# Autodesk Inventor assembly: 200-40-BOGIE-CONNECTOR-ASM-01
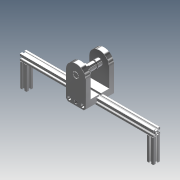
[picture p0: Inventor's stored thumbnail of the model, 180x180]
Saved by Autodesk Inventor 2018.2 (Build 222227000, 227)
## iProperties
Manager: feesmrt
Company: FRANC0R
Created: 2017-12-10
Part Number: 200-40-BOGIE-CONNECTOR-ASM-01
Material: Generisch
Document SubType Name: Assembly
Designer: feesmrt
Project: Rescue Robot
Cost Center: -
Description: Bogie Connector Assembly
Engineer: feesmrt
Authority: feesmrt
Stock Number: 200-40-BOGIE-CONNECTOR-ASM-01
Author: feesmrt
Title: Bogie Connector Assembly
Subject: Rescue Robot
Revision Number: 1
## Documents named in this file (10)
- D:\Programmierung\FRANC0R\CAD\02-Rocker-Bogie-Robot\200-ROCKER-BOGIE\200-40-BOGIE-CONNECTOR-ASM-01.iam
- D:\Programmierung\FRANC0R\CAD\02-Rocker-Bogie-Robot\900-COMPONENTS\900-50-PROFILES\90-50-PROFILES-20x20x400.ipt
- D:\Programmierung\FRANC0R\CAD\02-Rocker-Bogie-Robot\900-COMPONENTS\900-50-PROFILES\90-50-PROFILES-20x20x70.ipt
- D:\Programmierung\FRANC0R\CAD\02-Rocker-Bogie-Robot\200-ROCKER-BOGIE\200-40-BOGIE-CONNECTOR-05.ipt
- D:\Programmierung\FRANC0R\CAD\02-Rocker-Bogie-Robot\200-ROCKER-BOGIE\200-40-BOGIE-CONNECTOR-03.ipt
- D:\Programmierung\FRANC0R\CAD\02-Rocker-Bogie-Robot\200-ROCKER-BOGIE\200-40-BOGIE-CONNECTOR-04.ipt
- D:\Programmierung\FRANC0R\CAD\02-Rocker-Bogie-Robot\900-COMPONENTS\900-40-SCREWS\900-40-SCREWS-DIN7984_M5x25.ipt
- D:\Programmierung\FRANC0R\CAD\02-Rocker-Bogie-Robot\900-COMPONENTS\900-40-SCREWS\900-40-SCREWS-DIN7984_M5x12.ipt
- D:\Programmierung\FRANC0R\CAD\02-Rocker-Bogie-Robot\900-COMPONENTS\900-50-PROFILES\900-50-PROFILES-CONN-N6xM5.ipt
- D:\Programmierung\FRANC0R\CAD\02-Rocker-Bogie-Robot\900-COMPONENTS\900-60-CIRCLIPS\900-60-CIRCLIPS-DIN471-20x1,2.ipt
## Components (19 placed, 9 different names)
1. 200-40-BOGIE-CONNECTOR-05:1 — Passend:6, Passend:7, Fluchtend:7, Passend:8, Passend:9, Passend:10, Passend:45, Passend:46
2. 200-40-BOGIE-CONNECTOR-03:2 — Passend:8, Passend:9, Passend:10, Passend:16, Fluchtend:10, Passend:23, Passend:25, Passend:34, Passend:35
3. 200-40-BOGIE-CONNECTOR-03:1 — Passend:6, Passend:7, Fluchtend:7, Passend:17, Passend:24, Fluchtend:11, Passend:33, Passend:36
4. 90-50-PROFILES-20x20x400:1 — Passend:4, Fluchtend:3, Fluchtend:4, Passend:5, Fluchtend:5, Fluchtend:6, Fluchtend:9, Passend:21, Passend:22
5. 90-50-PROFILES-20x20x70:1 — Passend:5, Fluchtend:5, Fluchtend:6
6. 90-50-PROFILES-20x20x70:2 — Passend:4, Fluchtend:3, Fluchtend:4
7. 200-40-BOGIE-CONNECTOR-04:1 — Passend:17, Passend:21, Passend:24, Fluchtend:11, Passend:29, Passend:30, Passend:31, Passend:32, Passend:39, Passend:40, Winkel:1, Winkel:2
8. 200-40-BOGIE-CONNECTOR-04:2 — Passend:16, Passend:22, Fluchtend:10, Passend:23, Passend:26, Passend:27, Passend:28, Passend:37, Passend:38, Winkel:3, Winkel:4
9. 900-40-SCREWS-DIN7984_M5x25:1 — Passend:25, Passend:26, Passend:41
10. 900-40-SCREWS-DIN7984_M5x25:2 — Passend:27, Passend:28, Passend:42
11. 900-40-SCREWS-DIN7984_M5x25:3 — Passend:30, Passend:32, Passend:44
12. 900-40-SCREWS-DIN7984_M5x25:4 — Passend:29, Passend:31, Passend:43
13. 900-40-SCREWS-DIN7984_M5x12:1 — Passend:33, Passend:36
14. 900-40-SCREWS-DIN7984_M5x12:2 — Passend:34, Passend:35
15. 900-50-PROFILES-CONN-N6xM5:1 — Passend:37, Passend:42, Winkel:4
16. 900-50-PROFILES-CONN-N6xM5:2 — Passend:38, Passend:41, Winkel:3
17. 900-50-PROFILES-CONN-N6xM5:3 — Passend:40, Passend:44, Winkel:2
18. 900-50-PROFILES-CONN-N6xM5:4 — Passend:39, Passend:43, Winkel:1
19. 900-60-CIRCLIPS-DIN471-20x1,2:1 — Passend:45, Passend:46, Fluchtend:12
## Relationships (48: Mate 35, Flush 9, Angle 4)
- Passend:4 [Mate]: 90-50-PROFILES-20x20x400:1 ↔ 90-50-PROFILES-20x20x70:2
- Fluchtend:3 [Flush]: 90-50-PROFILES-20x20x400:1 ↔ 90-50-PROFILES-20x20x70:2
- Fluchtend:4 [Flush]: 90-50-PROFILES-20x20x400:1 ↔ 90-50-PROFILES-20x20x70:2
- Passend:5 [Mate]: 90-50-PROFILES-20x20x400:1 ↔ 90-50-PROFILES-20x20x70:1
- Fluchtend:5 [Flush]: 90-50-PROFILES-20x20x400:1 ↔ 90-50-PROFILES-20x20x70:1
- Fluchtend:6 [Flush]: 90-50-PROFILES-20x20x400:1 ↔ 90-50-PROFILES-20x20x70:1
- Passend:6 [Mate]: 200-40-BOGIE-CONNECTOR-05:1 ↔ 200-40-BOGIE-CONNECTOR-03:1
- Passend:7 [Mate]: 200-40-BOGIE-CONNECTOR-05:1 ↔ 200-40-BOGIE-CONNECTOR-03:1
- Fluchtend:7 [Flush]: 200-40-BOGIE-CONNECTOR-05:1 ↔ 200-40-BOGIE-CONNECTOR-03:1
- Passend:8 [Mate]: 200-40-BOGIE-CONNECTOR-05:1 ↔ 200-40-BOGIE-CONNECTOR-03:2
- Passend:9 [Mate]: 200-40-BOGIE-CONNECTOR-05:1 ↔ 200-40-BOGIE-CONNECTOR-03:2
- Passend:10 [Mate]: 200-40-BOGIE-CONNECTOR-05:1 ↔ 200-40-BOGIE-CONNECTOR-03:2
- Passend:16 [Mate]: 200-40-BOGIE-CONNECTOR-03:2 ↔ 200-40-BOGIE-CONNECTOR-04:2
- Fluchtend:9 [Flush]: 90-50-PROFILES-20x20x400:1
- Passend:17 [Mate]: 200-40-BOGIE-CONNECTOR-03:1 ↔ 200-40-BOGIE-CONNECTOR-04:1
- Passend:21 [Mate]: 90-50-PROFILES-20x20x400:1 ↔ 200-40-BOGIE-CONNECTOR-04:1
- Passend:22 [Mate]: 90-50-PROFILES-20x20x400:1 ↔ 200-40-BOGIE-CONNECTOR-04:2
- Fluchtend:10 [Flush]: 200-40-BOGIE-CONNECTOR-03:2 ↔ 200-40-BOGIE-CONNECTOR-04:2
- Passend:23 [Mate]: 200-40-BOGIE-CONNECTOR-03:2 ↔ 200-40-BOGIE-CONNECTOR-04:2
- Passend:24 [Mate]: 200-40-BOGIE-CONNECTOR-03:1 ↔ 200-40-BOGIE-CONNECTOR-04:1
- Fluchtend:11 [Flush]: 200-40-BOGIE-CONNECTOR-03:1 ↔ 200-40-BOGIE-CONNECTOR-04:1
- Passend:25 [Mate]: 200-40-BOGIE-CONNECTOR-03:2 ↔ 900-40-SCREWS-DIN7984_M5x25:1
- Passend:26 [Mate]: 200-40-BOGIE-CONNECTOR-04:2 ↔ 900-40-SCREWS-DIN7984_M5x25:1
- Passend:27 [Mate]: 200-40-BOGIE-CONNECTOR-04:2 ↔ 900-40-SCREWS-DIN7984_M5x25:2
- Passend:28 [Mate]: 200-40-BOGIE-CONNECTOR-04:2 ↔ 900-40-SCREWS-DIN7984_M5x25:2
- Passend:29 [Mate]: 200-40-BOGIE-CONNECTOR-04:1 ↔ 900-40-SCREWS-DIN7984_M5x25:4
- Passend:30 [Mate]: 200-40-BOGIE-CONNECTOR-04:1 ↔ 900-40-SCREWS-DIN7984_M5x25:3
- Passend:31 [Mate]: 200-40-BOGIE-CONNECTOR-04:1 ↔ 900-40-SCREWS-DIN7984_M5x25:4
- Passend:32 [Mate]: 200-40-BOGIE-CONNECTOR-04:1 ↔ 900-40-SCREWS-DIN7984_M5x25:3
- Passend:33 [Mate]: 200-40-BOGIE-CONNECTOR-03:1 ↔ 900-40-SCREWS-DIN7984_M5x12:1
- Passend:34 [Mate]: 200-40-BOGIE-CONNECTOR-03:2 ↔ 900-40-SCREWS-DIN7984_M5x12:2
- Passend:35 [Mate]: 200-40-BOGIE-CONNECTOR-03:2 ↔ 900-40-SCREWS-DIN7984_M5x12:2
- Passend:36 [Mate]: 200-40-BOGIE-CONNECTOR-03:1 ↔ 900-40-SCREWS-DIN7984_M5x12:1
- Passend:37 [Mate] (1.5 mm): 200-40-BOGIE-CONNECTOR-04:2 ↔ 900-50-PROFILES-CONN-N6xM5:1
- Passend:38 [Mate] (1.5 mm): 200-40-BOGIE-CONNECTOR-04:2 ↔ 900-50-PROFILES-CONN-N6xM5:2
- Passend:39 [Mate] (1.5 mm): 200-40-BOGIE-CONNECTOR-04:1 ↔ 900-50-PROFILES-CONN-N6xM5:4
- Passend:40 [Mate] (1.5 mm): 200-40-BOGIE-CONNECTOR-04:1 ↔ 900-50-PROFILES-CONN-N6xM5:3
- Passend:41 [Mate]: 900-40-SCREWS-DIN7984_M5x25:1 ↔ 900-50-PROFILES-CONN-N6xM5:2
- Passend:42 [Mate]: 900-40-SCREWS-DIN7984_M5x25:2 ↔ 900-50-PROFILES-CONN-N6xM5:1
- Passend:43 [Mate]: 900-40-SCREWS-DIN7984_M5x25:4 ↔ 900-50-PROFILES-CONN-N6xM5:4
- Passend:44 [Mate]: 900-40-SCREWS-DIN7984_M5x25:3 ↔ 900-50-PROFILES-CONN-N6xM5:3
- Winkel:1 [Angle] (0 deg): 200-40-BOGIE-CONNECTOR-04:1 ↔ 900-50-PROFILES-CONN-N6xM5:4
- Winkel:2 [Angle] (0 deg): 200-40-BOGIE-CONNECTOR-04:1 ↔ 900-50-PROFILES-CONN-N6xM5:3
- Winkel:3 [Angle] (0 deg): 200-40-BOGIE-CONNECTOR-04:2 ↔ 900-50-PROFILES-CONN-N6xM5:2
- Winkel:4 [Angle] (0 deg): 200-40-BOGIE-CONNECTOR-04:2 ↔ 900-50-PROFILES-CONN-N6xM5:1
- Passend:45 [Mate]: 200-40-BOGIE-CONNECTOR-05:1 ↔ 900-60-CIRCLIPS-DIN471-20x1,2:1
- Passend:46 [Mate]: 200-40-BOGIE-CONNECTOR-05:1 ↔ 900-60-CIRCLIPS-DIN471-20x1,2:1
- Fluchtend:12 [Flush]: 900-60-CIRCLIPS-DIN471-20x1,2:1
